# Autodesk Inventor assembly: Overall_Assembly_Rev3
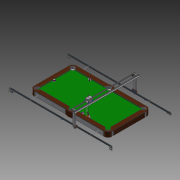
[picture p0: Inventor's stored thumbnail of the model, 180x180]
Saved by Autodesk Inventor 2015 (Build 190159000, 159)
## iProperties
Created: 2017-01-22
Part Number: Overall_Assembly_Rev3
Document SubType Name: Assembly
Designer: Guy
Author: Guy
## Documents named in this file (8)
- C:\Users\Guy\Documents\Fourth Year\Capstone\git\Capstone-Project\doc\CAD\LowLevel_Rev3\Overall_Assembly_Rev3.iam
- C:\Users\Guy\Documents\Fourth Year\Capstone\git\Capstone-Project\doc\CAD\Pool Table\Table_Model.ipt
- C:\Users\Guy\Documents\Fourth Year\Capstone\git\Capstone-Project\doc\CAD\LowLevel_Rev3\X_rail_Assembly_Rev3.iam
- C:\Users\Guy\Documents\Fourth Year\Capstone\git\Capstone-Project\doc\CAD\LowLevel_Rev3\Y_rail_Assembly_Rev3.iam
- C:\Users\Guy\Documents\Fourth Year\Capstone\git\Capstone-Project\doc\CAD\LowLevel_Rev2\Pool_Ball_Stripe.ipt
- C:\Users\Guy\Documents\Fourth Year\Capstone\git\Capstone-Project\doc\CAD\Nuts and Bolts\1-2in_13tpi x 8 in.ipt
- C:\Users\Guy\Documents\Fourth Year\Capstone\git\Capstone-Project\doc\CAD\SM2\Overall_Shooting_Mechanism2.iam
- C:\Users\Guy\Documents\Fourth Year\Capstone\git\Capstone-Project\doc\CAD\Stepper Motor\NEMA-17\NEMA 17 with T5 Pulley.iam
## Components (13 placed, 7 different names)
1. Table_Model:1 — Tangent:1, Tangent:2, Tangent:3, Tangent:4, Tangent:5, Tangent:6, Mate:49, Mate:52, Mate:57, Mate:58, Mate:80, Mate:83, Tangent:7, Angle:1
2. Pool_Ball_Stripe:1 — Tangent:1, Tangent:2
3. Pool_Ball_Stripe:2 — Tangent:3, Tangent:4
4. Pool_Ball_Stripe:3 — Tangent:5, Tangent:6
5. 1-2in_13tpi x 8 in:1 — Mate:57, Mate:71, Mate:81
6. 1-2in_13tpi x 8 in:2 — Mate:58, Mate:69, Mate:70
7. 1-2in_13tpi x 8 in:3 — Mate:49, Mate:76, Mate:77
8. 1-2in_13tpi x 8 in:4 — Mate:52, Mate:74, Mate:75
9. X_rail_Assembly_Rev3:1 [sub-assembly] — Mate:69, Mate:70, Mate:71, Mate:80, Mate:81, Flush:1, Mate:85, Mate:91, Mate:92, Mate:93, Mate:94
10. X_rail_Assembly_Rev3:2 [sub-assembly] — Mate:74, Mate:75, Mate:76, Mate:77, Mate:83, Angle:1, Flush:1, Mate:86, Mate:89, Flush:2
11. Overall_Shooting_Mechanism2:1 [sub-assembly] — Tangent:7, Mate:90
12. Y_rail_Assembly_Rev3:1 [sub-assembly] — Mate:85, Mate:86, Mate:88, Mate:90, Mate:91, Mate:92, Mate:93, Mate:94
13. NEMA 17 with T5 Pulley:1 [sub-assembly] — Mate:88, Mate:89, Flush:2
## Relationships (33: Mate 23, Tangent 7, Flush 2, Angle 1)
- Tangent:1: Table_Model:1 ↔ Pool_Ball_Stripe:1
- Tangent:2: Table_Model:1 ↔ Pool_Ball_Stripe:1
- Tangent:3: Table_Model:1 ↔ Pool_Ball_Stripe:2
- Tangent:4: Table_Model:1 ↔ Pool_Ball_Stripe:2
- Tangent:5: Table_Model:1 ↔ Pool_Ball_Stripe:3
- Tangent:6: Table_Model:1 ↔ Pool_Ball_Stripe:3
- Mate:49: Table_Model:1 ↔ 1-2in_13tpi x 8 in:3
- Mate:52: Table_Model:1 ↔ 1-2in_13tpi x 8 in:4
- Mate:57: Table_Model:1 ↔ 1-2in_13tpi x 8 in:1
- Mate:58: Table_Model:1 ↔ 1-2in_13tpi x 8 in:2
- Mate:69: 1-2in_13tpi x 8 in:2 ↔ X_rail_Assembly_Rev3:1
- Mate:70: 1-2in_13tpi x 8 in:2 ↔ X_rail_Assembly_Rev3:1
- Mate:71: 1-2in_13tpi x 8 in:1 ↔ X_rail_Assembly_Rev3:1
- Mate:74: 1-2in_13tpi x 8 in:4 ↔ X_rail_Assembly_Rev3:2
- Mate:75: 1-2in_13tpi x 8 in:4 ↔ X_rail_Assembly_Rev3:2
- Mate:76: 1-2in_13tpi x 8 in:3 ↔ X_rail_Assembly_Rev3:2
- Mate:77: 1-2in_13tpi x 8 in:3 ↔ X_rail_Assembly_Rev3:2
- Mate:80 (220 mm): Table_Model:1 ↔ X_rail_Assembly_Rev3:1
- Mate:81: 1-2in_13tpi x 8 in:1 ↔ X_rail_Assembly_Rev3:1
- Mate:83 (201 mm): Table_Model:1 ↔ X_rail_Assembly_Rev3:2
- Tangent:7: Table_Model:1 ↔ Overall_Shooting_Mechanism2:1
- Angle:1 (0 deg): Table_Model:1 ↔ X_rail_Assembly_Rev3:2
- Flush:1: X_rail_Assembly_Rev3:1 ↔ X_rail_Assembly_Rev3:2
- Mate:85: X_rail_Assembly_Rev3:1 ↔ Y_rail_Assembly_Rev3:1
- Mate:86: X_rail_Assembly_Rev3:2 ↔ Y_rail_Assembly_Rev3:1
- Mate:88: Y_rail_Assembly_Rev3:1 ↔ NEMA 17 with T5 Pulley:1
- Mate:89: X_rail_Assembly_Rev3:2 ↔ NEMA 17 with T5 Pulley:1
- Flush:2: X_rail_Assembly_Rev3:2 ↔ NEMA 17 with T5 Pulley:1
- Mate:90: Overall_Shooting_Mechanism2:1 ↔ Y_rail_Assembly_Rev3:1
- Mate:91: X_rail_Assembly_Rev3:1 ↔ Y_rail_Assembly_Rev3:1
- Mate:92: X_rail_Assembly_Rev3:1 ↔ Y_rail_Assembly_Rev3:1
- Mate:93: X_rail_Assembly_Rev3:1 ↔ Y_rail_Assembly_Rev3:1
- Mate:94: X_rail_Assembly_Rev3:1 ↔ Y_rail_Assembly_Rev3:1
